# Autodesk Inventor assembly: ASY Мешалка 2.0
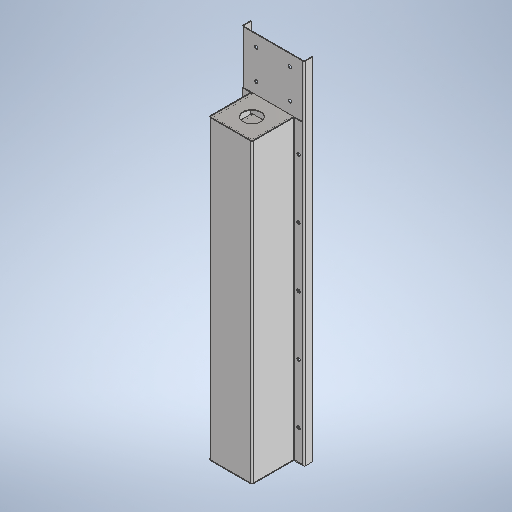
[picture p0: Inventor's stored thumbnail of the model, 512x512]
Saved by Autodesk Inventor 2025 (Build 290162010, 162A)
## iProperties
Created: 2024-04-16
Part Number: ASY Мешалка 2.0
Document SubType Name: Assembly
Designer: pokla
Author: pokla
## Documents named in this file (7)
- C:\Users\pokla\Documents\Inventor\Мешалка\ASY Мешалка 2.0.iam
- C:\Users\pokla\Documents\Inventor\Мешалка\Новые детали\Крепление 2.0.ipt
- C:\Users\pokla\Documents\Inventor\Мешалка\Новые детали\Крепление корпуса 2.0.ipt
- C:\Users\pokla\Documents\Inventor\Мешалка\Новые детали\Параметры.ipt
- C:\Users\pokla\Documents\Inventor\Мешалка\Кожух.ipt
- C:\Users\pokla\Documents\Inventor\Мешалка\Опоры на кожухе.ipt
- C:\Users\pokla\Documents\Inventor\Мешалка\Опоры на кожухе 2.ipt
## Components (11 placed, 6 different names)
1. Крепление 2.0:1 — Flush:1, Mate:1, Rigid:2, Rigid:3, Rigid:7, Rigid:8
2. Крепление корпуса 2.0:2 — Rigid:3
3. Крепление корпуса 2.0:3 — Rigid:2, Rigid:4
4. Параметры:1
5. Кожух:1 — Rigid:4, Rigid:5, Rigid:6, Rigid:9, Rigid:10
6. Опоры на кожухе:1 — Rigid:5
7. Опоры на кожухе 2:1 — Rigid:6
8. Крепление корпуса 2.0:4 — Rigid:7
9. Крепление корпуса 2.0:5 — Rigid:8
10. Опоры на кожухе 2:2 — Rigid:9
11. Опоры на кожухе 2:3 — Rigid:10
## Relationships (11: WeldJoint 9, Flush 1, Mate 1)
- Flush:1: Крепление 2.0:1
- Mate:1: Крепление 2.0:1
- Rigid:2 [WeldJoint] (-150 mm): Крепление 2.0:1 ↔ Крепление корпуса 2.0:3
- Rigid:3 [WeldJoint] (-5 mm): Крепление 2.0:1 ↔ Крепление корпуса 2.0:2
- Rigid:4 [WeldJoint]: Крепление корпуса 2.0:3 ↔ Кожух:1
- Rigid:5 [WeldJoint]: Кожух:1 ↔ Опоры на кожухе:1
- Rigid:6 [WeldJoint] (-2 mm): Кожух:1 ↔ Опоры на кожухе 2:1
- Rigid:7 [WeldJoint] (-202 mm): Крепление 2.0:1 ↔ Крепление корпуса 2.0:4
- Rigid:8 [WeldJoint] (-52 mm): Крепление 2.0:1 ↔ Крепление корпуса 2.0:5
- Rigid:9 [WeldJoint] (-54 mm): Кожух:1 ↔ Опоры на кожухе 2:2
- Rigid:10 [WeldJoint] (-45 mm): Кожух:1 ↔ Опоры на кожухе 2:3
